# Autodesk Inventor assembly: КВ33.044.000
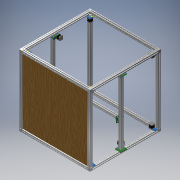
[picture p0: Inventor's stored thumbnail of the model, 180x180]
Saved by Autodesk Inventor 2019 (Build 230136000, 136)
## iProperties
Created: 2019-07-15
Part Number: КВ33.044.000
Material: Типовые
Document SubType Name: Assembly
Designer: Петров Иван
Description: Сортирующая ячейка
Author: Петров Иван
## Documents named in this file (8)
- C:\Users\user\Documents\Kvantoriada2019\optimal_gripper\hardware\КВ33.044.000 - Сортирующая ячейка.iam
- C:\Users\user\Documents\Kvantoriada2019\optimal_gripper\hardware\Стандартные изделия\Профиль станочный 30x30x740.ipt
- C:\Users\user\Documents\Kvantoriada2019\optimal_gripper\hardware\Стандартные изделия\Угол соединительный 30х30х30.ipt
- C:\Users\user\Documents\Kvantoriada2019\optimal_gripper\hardware\КВ33.044.200 - Каретка оси Х.iam
- C:\Users\user\Documents\Kvantoriada2019\optimal_gripper\hardware\Стандартные изделия\Профиль станочный 30x30x728.ipt
- C:\Users\user\Documents\Kvantoriada2019\optimal_gripper\hardware\КВ33.044.001 - Дно.ipt
- C:\Users\user\Documents\Kvantoriada2019\optimal_gripper\hardware\КВ33.044.300 -  Сборка мотора Makeblock с крепление.iam
- C:\Users\user\Documents\Kvantoriada2019\optimal_gripper\hardware\КВ33.044.400 - Сборка деражтеля катка 6 мм.iam
## Components (45 placed, 7 different names)
1. Профиль станочный 30x30x740:1 — Заподлицо:9, Заподлицо:10, Совмещение:4, Заподлицо:12, Совмещение:9, Заподлицо:17
2. Профиль станочный 30x30x740:2 — Совмещение:3, Заподлицо:2, Заподлицо:3, Совмещение:66, Совмещение:67, Совмещение:105
3. Профиль станочный 30x30x740:3 — Совмещение:1, Заподлицо:1, Заподлицо:5, Заподлицо:6, Заподлицо:8, Совмещение:5, Совмещение:65, Совмещение:109
4. Профиль станочный 30x30x740:4 — Заподлицо:14, Совмещение:7, Заподлицо:16, Заподлицо:18, Заподлицо:19, Совмещение:10, Совмещение:100, Совмещение:113
5. Угол соединительный 30х30х30:1 — Совмещение:1, Совмещение:2, Совмещение:3, Заподлицо:1, Заподлицо:2, Заподлицо:3, Заподлицо:4, Заподлицо:5, Заподлицо:38
6. Угол соединительный 30х30х30:2 — Заподлицо:18, Заподлицо:19, Совмещение:10, Совмещение:11, Заподлицо:20, Заподлицо:21
7. Угол соединительный 30х30х30:3 — Заподлицо:6, Заподлицо:7, Заподлицо:8, Заподлицо:9, Заподлицо:10, Совмещение:4, Заподлицо:11, Совмещение:5, Совмещение:6
8. Угол соединительный 30х30х30:4 — Заподлицо:12, Заподлицо:13, Заподлицо:14, Заподлицо:15, Совмещение:7, Совмещение:8, Заподлицо:16, Совмещение:9, Заподлицо:17
9. Профиль станочный 30x30x740:9 — Заподлицо:7, Заподлицо:11, Совмещение:6, Совмещение:19, Заподлицо:36, Заподлицо:37, Совмещение:58, Касательность:20, Касательность:21, Совмещение:106, Заподлицо:45, Совмещение:108, Заподлицо:46
10. Профиль станочный 30x30x740:10 — Заподлицо:13, Заподлицо:15, Совмещение:8, Совмещение:110, Заподлицо:47, Совмещение:112, Заподлицо:48
11. Профиль станочный 30x30x740:11 — Совмещение:11, Заподлицо:20, Заподлицо:21, Совмещение:98, Заподлицо:41, Совмещение:101, Заподлицо:42
12. Профиль станочный 30x30x740:12 — Совмещение:2, Заподлицо:4, Заподлицо:38, Совмещение:51, Касательность:18, Касательность:19, Совмещение:102, Заподлицо:43, Совмещение:104, Заподлицо:44
13. Профиль станочный 30x30x740:15
14. Профиль станочный 30x30x740:16
15. Профиль станочный 30x30x740:17 — Совмещение:103, Совмещение:107
16. Профиль станочный 30x30x740:18 — Совмещение:99, Совмещение:111
17. Угол соединительный 30х30х30:5
18. Угол соединительный 30х30х30:6
19. Угол соединительный 30х30х30:7 — Совмещение:19, Заподлицо:36, Заподлицо:37
20. Угол соединительный 30х30х30:8
21. КВ33.044.200 - Каретка оси Х:6 [sub-assembly] — Совмещение:42, Совмещение:59, Совмещение:60, Совмещение:64, Касательность:22, Касательность:23, Совмещение:119
22. КВ33.044.200 - Каретка оси Х:7 [sub-assembly] — Совмещение:61, Совмещение:62, Совмещение:63, Касательность:24, Совмещение:125
23. Профиль станочный 30x30x728:4 — Совмещение:41, Касательность:16, Касательность:17, Совмещение:42, Совмещение:59, Совмещение:60, Совмещение:61, Совмещение:62, Совмещение:63, Совмещение:118, Заподлицо:119, Совмещение:124, Заподлицо:122
24. КВ33.044.200 - Каретка оси Х:8 [sub-assembly] — Совмещение:41, Касательность:16, Касательность:17
25. КВ33.044.200 - Каретка оси Х:9 [sub-assembly] — Совмещение:44, Совмещение:45, Совмещение:46, Совмещение:51, Касательность:18, Касательность:19, Совмещение:117
26. КВ33.044.200 - Каретка оси Х:10 [sub-assembly] — Совмещение:48, Совмещение:49, Совмещение:50, Совмещение:123
27. Профиль станочный 30x30x728:5 — Совмещение:44, Совмещение:45, Совмещение:46, Совмещение:48, Совмещение:49, Совмещение:50, Совмещение:64, Касательность:22, Касательность:23, Совмещение:116, Заподлицо:118, Совмещение:122, Заподлицо:121
28. КВ33.044.200 - Каретка оси Х:11 [sub-assembly] — Совмещение:58, Касательность:20, Касательность:21, Совмещение:121
29. КВ33.044.200 - Каретка оси Х:12 [sub-assembly] — Совмещение:115
30. Профиль станочный 30x30x728:6 — Касательность:24, Совмещение:114, Заподлицо:49, Совмещение:120, Заподлицо:120
31. КВ33.044.001 - Дно:1 — Совмещение:65, Совмещение:66, Совмещение:67
32. КВ33.044.400 - Сборка деражтеля катка 6 мм:6 [sub-assembly] — Совмещение:100, Совмещение:101, Заподлицо:42
33. КВ33.044.300 -  Сборка мотора Makeblock с крепление:3 [sub-assembly] — Совмещение:98, Совмещение:99, Заподлицо:41
34. КВ33.044.300 -  Сборка мотора Makeblock с крепление:4 [sub-assembly] — Совмещение:102, Заподлицо:43, Совмещение:103
35. КВ33.044.300 -  Сборка мотора Makeblock с крепление:5 [sub-assembly] — Совмещение:110, Заподлицо:47, Совмещение:111
36. КВ33.044.300 -  Сборка мотора Makeblock с крепление:6 [sub-assembly] — Совмещение:106, Совмещение:107, Заподлицо:45
37. КВ33.044.400 - Сборка деражтеля катка 6 мм:7 [sub-assembly] — Совмещение:104, Заподлицо:44, Совмещение:105
38. КВ33.044.400 - Сборка деражтеля катка 6 мм:9 [sub-assembly] — Совмещение:108, Совмещение:109, Заподлицо:46
39. КВ33.044.400 - Сборка деражтеля катка 6 мм:10 [sub-assembly] — Совмещение:112, Заподлицо:48, Совмещение:113
40. КВ33.044.300 -  Сборка мотора Makeblock с крепление:7 [sub-assembly] — Совмещение:114, Совмещение:115, Заподлицо:49
41. КВ33.044.300 -  Сборка мотора Makeblock с крепление:8 [sub-assembly] — Совмещение:116, Заподлицо:118, Совмещение:117
42. КВ33.044.300 -  Сборка мотора Makeblock с крепление:9 [sub-assembly] — Совмещение:118, Заподлицо:119, Совмещение:119
43. КВ33.044.400 - Сборка деражтеля катка 6 мм:11 [sub-assembly] — Совмещение:120, Совмещение:121, Заподлицо:120
44. КВ33.044.400 - Сборка деражтеля катка 6 мм:12 [sub-assembly] — Совмещение:122, Совмещение:123, Заподлицо:121
45. КВ33.044.400 - Сборка деражтеля катка 6 мм:13 [sub-assembly] — Совмещение:124, Совмещение:125, Заподлицо:122
## Relationships (133: Mate 72, Flush 52, Tangent 9)
- Совмещение:1 [Mate]: Профиль станочный 30x30x740:3 ↔ Угол соединительный 30х30х30:1
- Совмещение:2 [Mate]: Угол соединительный 30х30х30:1 ↔ Профиль станочный 30x30x740:12
- Совмещение:3 [Mate]: Профиль станочный 30x30x740:2 ↔ Угол соединительный 30х30х30:1
- Заподлицо:1 [Flush]: Профиль станочный 30x30x740:3 ↔ Угол соединительный 30х30х30:1
- Заподлицо:2 [Flush]: Профиль станочный 30x30x740:2 ↔ Угол соединительный 30х30х30:1
- Заподлицо:3 [Flush]: Профиль станочный 30x30x740:2 ↔ Угол соединительный 30х30х30:1
- Заподлицо:4 [Flush]: Угол соединительный 30х30х30:1 ↔ Профиль станочный 30x30x740:12
- Заподлицо:5 [Flush]: Профиль станочный 30x30x740:3 ↔ Угол соединительный 30х30х30:1
- Заподлицо:6 [Flush]: Профиль станочный 30x30x740:3 ↔ Угол соединительный 30х30х30:3
- Заподлицо:7 [Flush]: Угол соединительный 30х30х30:3 ↔ Профиль станочный 30x30x740:9
- Заподлицо:8 [Flush]: Профиль станочный 30x30x740:3 ↔ Угол соединительный 30х30х30:3
- Заподлицо:9 [Flush]: Профиль станочный 30x30x740:1 ↔ Угол соединительный 30х30х30:3
- Заподлицо:10 [Flush]: Профиль станочный 30x30x740:1 ↔ Угол соединительный 30х30х30:3
- Совмещение:4 [Mate]: Профиль станочный 30x30x740:1 ↔ Угол соединительный 30х30х30:3
- Заподлицо:11 [Flush]: Угол соединительный 30х30х30:3 ↔ Профиль станочный 30x30x740:9
- Совмещение:5 [Mate]: Профиль станочный 30x30x740:3 ↔ Угол соединительный 30х30х30:3
- Совмещение:6 [Mate]: Угол соединительный 30х30х30:3 ↔ Профиль станочный 30x30x740:9
- Заподлицо:12 [Flush]: Профиль станочный 30x30x740:1 ↔ Угол соединительный 30х30х30:4
- Заподлицо:13 [Flush]: Угол соединительный 30х30х30:4 ↔ Профиль станочный 30x30x740:10
- Заподлицо:14 [Flush]: Профиль станочный 30x30x740:4 ↔ Угол соединительный 30х30х30:4
- Заподлицо:15 [Flush]: Угол соединительный 30х30х30:4 ↔ Профиль станочный 30x30x740:10
- Совмещение:7 [Mate]: Профиль станочный 30x30x740:4 ↔ Угол соединительный 30х30х30:4
- Совмещение:8 [Mate]: Угол соединительный 30х30х30:4 ↔ Профиль станочный 30x30x740:10
- Заподлицо:16 [Flush]: Профиль станочный 30x30x740:4 ↔ Угол соединительный 30х30х30:4
- Совмещение:9 [Mate]: Профиль станочный 30x30x740:1 ↔ Угол соединительный 30х30х30:4
- Заподлицо:17 [Flush]: Профиль станочный 30x30x740:1 ↔ Угол соединительный 30х30х30:4
- Заподлицо:18 [Flush]: Профиль станочный 30x30x740:4 ↔ Угол соединительный 30х30х30:2
- Заподлицо:19 [Flush]: Профиль станочный 30x30x740:4 ↔ Угол соединительный 30х30х30:2
- Совмещение:10 [Mate]: Профиль станочный 30x30x740:4 ↔ Угол соединительный 30х30х30:2
- Совмещение:11 [Mate]: Угол соединительный 30х30х30:2 ↔ Профиль станочный 30x30x740:11
- Заподлицо:20 [Flush]: Угол соединительный 30х30х30:2 ↔ Профиль станочный 30x30x740:11
- Заподлицо:21 [Flush]: Угол соединительный 30х30х30:2 ↔ Профиль станочный 30x30x740:11
- [Mate]: Профиль станочный 30x30x740:17 ↔ Угол соединительный 30х30х30:5
- [Mate]: Профиль станочный 30x30x740:16 ↔ Угол соединительный 30х30х30:5
- [Flush]: Профиль станочный 30x30x740:17 ↔ Угол соединительный 30х30х30:5
- [Flush]: Профиль станочный 30x30x740:16 ↔ Угол соединительный 30х30х30:5
- [Flush]: Профиль станочный 30x30x740:16 ↔ Угол соединительный 30х30х30:5
- [Flush]: Профиль станочный 30x30x740:17 ↔ Угол соединительный 30х30х30:5
- [Flush]: Профиль станочный 30x30x740:17 ↔ Угол соединительный 30х30х30:7
- [Flush]: Профиль станочный 30x30x740:17 ↔ Угол соединительный 30х30х30:7
- [Flush]: Профиль станочный 30x30x740:15 ↔ Угол соединительный 30х30х30:7
- [Flush]: Профиль станочный 30x30x740:15 ↔ Угол соединительный 30х30х30:7
- [Mate]: Профиль станочный 30x30x740:15 ↔ Угол соединительный 30х30х30:7
- [Mate]: Профиль станочный 30x30x740:17 ↔ Угол соединительный 30х30х30:7
- [Flush]: Профиль станочный 30x30x740:15 ↔ Угол соединительный 30х30х30:8
- [Flush]: Профиль станочный 30x30x740:18 ↔ Угол соединительный 30х30х30:8
- [Mate]: Профиль станочный 30x30x740:18 ↔ Угол соединительный 30х30х30:8
- [Flush]: Профиль станочный 30x30x740:18 ↔ Угол соединительный 30х30х30:8
- [Mate]: Профиль станочный 30x30x740:15 ↔ Угол соединительный 30х30х30:8
- [Flush]: Профиль станочный 30x30x740:15 ↔ Угол соединительный 30х30х30:8
- [Flush]: Профиль станочный 30x30x740:18 ↔ Угол соединительный 30х30х30:6
- [Flush]: Профиль станочный 30x30x740:18 ↔ Угол соединительный 30х30х30:6
- [Mate]: Профиль станочный 30x30x740:18 ↔ Угол соединительный 30х30х30:6
- Совмещение:19 [Mate]: Профиль станочный 30x30x740:9 ↔ Угол соединительный 30х30х30:7
- Заподлицо:36 [Flush]: Профиль станочный 30x30x740:9 ↔ Угол соединительный 30х30х30:7
- Заподлицо:37 [Flush]: Профиль станочный 30x30x740:9 ↔ Угол соединительный 30х30х30:7
- Заподлицо:38 [Flush]: Угол соединительный 30х30х30:1 ↔ Профиль станочный 30x30x740:12
- Совмещение:41 [Mate]: Профиль станочный 30x30x728:4 ↔ КВ33.044.200 - Каретка оси Х:8
- Касательность:16 [Tangent]: Профиль станочный 30x30x728:4 ↔ КВ33.044.200 - Каретка оси Х:8
- Касательность:17 [Tangent]: Профиль станочный 30x30x728:4 ↔ КВ33.044.200 - Каретка оси Х:8
- Совмещение:42 [Mate]: КВ33.044.200 - Каретка оси Х:6 ↔ Профиль станочный 30x30x728:4
- Совмещение:44 [Mate]: КВ33.044.200 - Каретка оси Х:9 ↔ Профиль станочный 30x30x728:5
- Совмещение:45 [Mate]: КВ33.044.200 - Каретка оси Х:9 ↔ Профиль станочный 30x30x728:5
- Совмещение:46 [Mate]: КВ33.044.200 - Каретка оси Х:9 ↔ Профиль станочный 30x30x728:5
- Совмещение:48 [Mate]: КВ33.044.200 - Каретка оси Х:10 ↔ Профиль станочный 30x30x728:5
- Совмещение:49 [Mate]: КВ33.044.200 - Каретка оси Х:10 ↔ Профиль станочный 30x30x728:5
- Совмещение:50 [Mate]: КВ33.044.200 - Каретка оси Х:10 ↔ Профиль станочный 30x30x728:5
- Совмещение:51 [Mate]: Профиль станочный 30x30x740:12 ↔ КВ33.044.200 - Каретка оси Х:9
- Касательность:18 [Tangent]: Профиль станочный 30x30x740:12 ↔ КВ33.044.200 - Каретка оси Х:9
- Касательность:19 [Tangent]: Профиль станочный 30x30x740:12 ↔ КВ33.044.200 - Каретка оси Х:9
- [Mate]: КВ33.044.200 - Каретка оси Х:11 ↔ Профиль станочный 30x30x728:6
- [Mate]: КВ33.044.200 - Каретка оси Х:11 ↔ Профиль станочный 30x30x728:6
- [Mate]: КВ33.044.200 - Каретка оси Х:11 ↔ Профиль станочный 30x30x728:6
- [Mate]: КВ33.044.200 - Каретка оси Х:12 ↔ Профиль станочный 30x30x728:6
- [Mate]: КВ33.044.200 - Каретка оси Х:12 ↔ Профиль станочный 30x30x728:6
- [Mate]: КВ33.044.200 - Каретка оси Х:12 ↔ Профиль станочный 30x30x728:6
- Совмещение:58 [Mate]: Профиль станочный 30x30x740:9 ↔ КВ33.044.200 - Каретка оси Х:11
- Касательность:20 [Tangent]: Профиль станочный 30x30x740:9 ↔ КВ33.044.200 - Каретка оси Х:11
- Касательность:21 [Tangent]: Профиль станочный 30x30x740:9 ↔ КВ33.044.200 - Каретка оси Х:11
- Совмещение:59 [Mate]: КВ33.044.200 - Каретка оси Х:6 ↔ Профиль станочный 30x30x728:4
- Совмещение:60 [Mate]: КВ33.044.200 - Каретка оси Х:6 ↔ Профиль станочный 30x30x728:4
- Совмещение:61 [Mate]: КВ33.044.200 - Каретка оси Х:7 ↔ Профиль станочный 30x30x728:4
- Совмещение:62 [Mate]: КВ33.044.200 - Каретка оси Х:7 ↔ Профиль станочный 30x30x728:4
- Совмещение:63 [Mate]: КВ33.044.200 - Каретка оси Х:7 ↔ Профиль станочный 30x30x728:4
- Совмещение:64 [Mate]: КВ33.044.200 - Каретка оси Х:6 ↔ Профиль станочный 30x30x728:5
- Касательность:22 [Tangent]: КВ33.044.200 - Каретка оси Х:6 ↔ Профиль станочный 30x30x728:5
- Касательность:23 [Tangent]: КВ33.044.200 - Каретка оси Х:6 ↔ Профиль станочный 30x30x728:5
- Касательность:24 [Tangent]: КВ33.044.200 - Каретка оси Х:7 ↔ Профиль станочный 30x30x728:6
- Совмещение:65 [Mate]: Профиль станочный 30x30x740:3 ↔ КВ33.044.001 - Дно:1
- Совмещение:66 [Mate]: Профиль станочный 30x30x740:2 ↔ КВ33.044.001 - Дно:1
- Совмещение:67 [Mate]: Профиль станочный 30x30x740:2 ↔ КВ33.044.001 - Дно:1
- Совмещение:98 [Mate]: Профиль станочный 30x30x740:11 ↔ КВ33.044.300 -  Сборка мотора Makeblock с крепление:3
- Совмещение:99 [Mate]: Профиль станочный 30x30x740:18 ↔ КВ33.044.300 -  Сборка мотора Makeblock с крепление:3
- Заподлицо:41 [Flush]: Профиль станочный 30x30x740:11 ↔ КВ33.044.300 -  Сборка мотора Makeblock с крепление:3
- Совмещение:100 [Mate]: Профиль станочный 30x30x740:4 ↔ КВ33.044.400 - Сборка деражтеля катка 6 мм:6
- Совмещение:101 [Mate]: Профиль станочный 30x30x740:11 ↔ КВ33.044.400 - Сборка деражтеля катка 6 мм:6
- Заподлицо:42 [Flush]: Профиль станочный 30x30x740:11 ↔ КВ33.044.400 - Сборка деражтеля катка 6 мм:6
- Совмещение:102 [Mate]: Профиль станочный 30x30x740:12 ↔ КВ33.044.300 -  Сборка мотора Makeblock с крепление:4
- Заподлицо:43 [Flush]: Профиль станочный 30x30x740:12 ↔ КВ33.044.300 -  Сборка мотора Makeblock с крепление:4
- Совмещение:103 [Mate]: Профиль станочный 30x30x740:17 ↔ КВ33.044.300 -  Сборка мотора Makeblock с крепление:4
- Совмещение:104 [Mate]: Профиль станочный 30x30x740:12 ↔ КВ33.044.400 - Сборка деражтеля катка 6 мм:7
- Заподлицо:44 [Flush]: Профиль станочный 30x30x740:12 ↔ КВ33.044.400 - Сборка деражтеля катка 6 мм:7
- Совмещение:105 [Mate]: Профиль станочный 30x30x740:2 ↔ КВ33.044.400 - Сборка деражтеля катка 6 мм:7
- Совмещение:106 [Mate]: Профиль станочный 30x30x740:9 ↔ КВ33.044.300 -  Сборка мотора Makeblock с крепление:6
- Совмещение:107 [Mate]: Профиль станочный 30x30x740:17 ↔ КВ33.044.300 -  Сборка мотора Makeblock с крепление:6
- Заподлицо:45 [Flush]: Профиль станочный 30x30x740:9 ↔ КВ33.044.300 -  Сборка мотора Makeblock с крепление:6
- Совмещение:108 [Mate]: Профиль станочный 30x30x740:9 ↔ КВ33.044.400 - Сборка деражтеля катка 6 мм:9
- Совмещение:109 [Mate]: Профиль станочный 30x30x740:3 ↔ КВ33.044.400 - Сборка деражтеля катка 6 мм:9
- Заподлицо:46 [Flush]: Профиль станочный 30x30x740:9 ↔ КВ33.044.400 - Сборка деражтеля катка 6 мм:9
- Совмещение:110 [Mate]: Профиль станочный 30x30x740:10 ↔ КВ33.044.300 -  Сборка мотора Makeblock с крепление:5
- Заподлицо:47 [Flush]: Профиль станочный 30x30x740:10 ↔ КВ33.044.300 -  Сборка мотора Makeblock с крепление:5
- Совмещение:111 [Mate]: Профиль станочный 30x30x740:18 ↔ КВ33.044.300 -  Сборка мотора Makeblock с крепление:5
- Совмещение:112 [Mate]: Профиль станочный 30x30x740:10 ↔ КВ33.044.400 - Сборка деражтеля катка 6 мм:10
- Заподлицо:48 [Flush]: Профиль станочный 30x30x740:10 ↔ КВ33.044.400 - Сборка деражтеля катка 6 мм:10
- Совмещение:113 [Mate]: Профиль станочный 30x30x740:4 ↔ КВ33.044.400 - Сборка деражтеля катка 6 мм:10
- Совмещение:114 [Mate]: Профиль станочный 30x30x728:6 ↔ КВ33.044.300 -  Сборка мотора Makeblock с крепление:7
- Совмещение:115 [Mate]: КВ33.044.200 - Каретка оси Х:12 ↔ КВ33.044.300 -  Сборка мотора Makeblock с крепление:7
- Заподлицо:49 [Flush]: Профиль станочный 30x30x728:6 ↔ КВ33.044.300 -  Сборка мотора Makeblock с крепление:7
- Совмещение:116 [Mate]: Профиль станочный 30x30x728:5 ↔ КВ33.044.300 -  Сборка мотора Makeblock с крепление:8
- Заподлицо:118 [Flush]: Профиль станочный 30x30x728:5 ↔ КВ33.044.300 -  Сборка мотора Makeblock с крепление:8
- Совмещение:117 [Mate]: КВ33.044.200 - Каретка оси Х:9 ↔ КВ33.044.300 -  Сборка мотора Makeblock с крепление:8
- Совмещение:118 [Mate]: Профиль станочный 30x30x728:4 ↔ КВ33.044.300 -  Сборка мотора Makeblock с крепление:9
- Заподлицо:119 [Flush]: Профиль станочный 30x30x728:4 ↔ КВ33.044.300 -  Сборка мотора Makeblock с крепление:9
- Совмещение:119 [Mate]: КВ33.044.200 - Каретка оси Х:6 ↔ КВ33.044.300 -  Сборка мотора Makeblock с крепление:9
- Совмещение:120 [Mate]: Профиль станочный 30x30x728:6 ↔ КВ33.044.400 - Сборка деражтеля катка 6 мм:11
- Совмещение:121 [Mate]: КВ33.044.200 - Каретка оси Х:11 ↔ КВ33.044.400 - Сборка деражтеля катка 6 мм:11
- Заподлицо:120 [Flush]: Профиль станочный 30x30x728:6 ↔ КВ33.044.400 - Сборка деражтеля катка 6 мм:11
- Совмещение:122 [Mate]: Профиль станочный 30x30x728:5 ↔ КВ33.044.400 - Сборка деражтеля катка 6 мм:12
- Совмещение:123 [Mate]: КВ33.044.200 - Каретка оси Х:10 ↔ КВ33.044.400 - Сборка деражтеля катка 6 мм:12
- Заподлицо:121 [Flush]: Профиль станочный 30x30x728:5 ↔ КВ33.044.400 - Сборка деражтеля катка 6 мм:12
- Совмещение:124 [Mate]: Профиль станочный 30x30x728:4 ↔ КВ33.044.400 - Сборка деражтеля катка 6 мм:13
- Совмещение:125 [Mate]: КВ33.044.200 - Каретка оси Х:7 ↔ КВ33.044.400 - Сборка деражтеля катка 6 мм:13
- Заподлицо:122 [Flush]: Профиль станочный 30x30x728:4 ↔ КВ33.044.400 - Сборка деражтеля катка 6 мм:13
## Named parameters: d91_d80 = 0 mm, d92_d82 = 0 mm, d93_d83 = 0 mm, d94_d84 = 0 mm, d95_d85 = 0 mm, d96_d86 = 0 mm, d97_d87 = 0 mm, d98_d66 = 0 mm, d99_d67 = 0 mm, d100_d69 = 0 mm, d101_d70 = 0 mm, d102_d71 = 0 mm, d103_d72 = 0 mm, d104_d74 = 0 mm, d105_d76 = 0 mm, d106_d78 = 0 mm, d107_d59 = 0 mm, d108_d61 = 0 mm, d109_d62 = 0 mm, d110_d63 = 0 mm, d111_d64 = 0 mm, d201_d189 = 0 mm, d202_d190 = 0 mm, d203_d191 = 0 mm, d204_d195 = 0 mm, d205_d196 = 0 mm, d206_d197 = 0 mm
